# Autodesk Inventor assembly: 20mm Camera Rig Assmebly For Robot
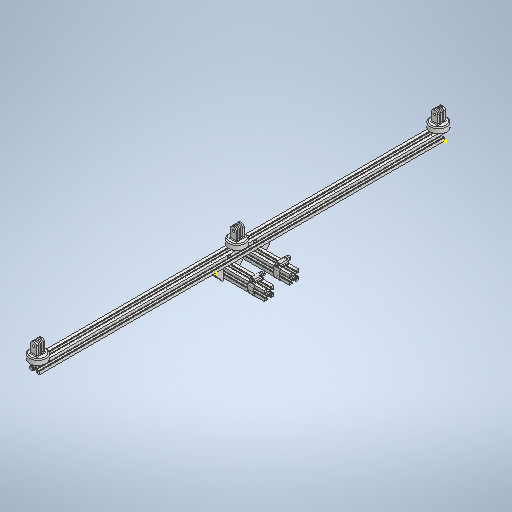
[picture p0: Inventor's stored thumbnail of the model, 512x512]
Saved by Autodesk Inventor 2025 (Build 290162010, 162A)
## iProperties
Created: 2024-07-24
Part Number: 20mm Camera Rig Assmebly For Robot
Document SubType Name: Assembly
Designer: Big Sean T
Author: Big Sean T
## Documents named in this file (9)
- D:\Underwater Camera RigScuba Resources\20mm Camera Rig Assmebly For Robot.iam
- D:\Underwater Camera RigScuba Resources\T slot beam 20mm.ipt
- D:\Underwater Camera RigScuba Resources\Go Pro Mount with threaded mount.ipt
- D:\Underwater Camera RigScuba Resources\M5 Model.ipt
- D:\Underwater Camera RigScuba Resources\90 Degree attachment T Slot.ipt
- D:\Underwater Camera RigScuba Resources\5mm Button Head Screw Botch.ipt
- D:\Underwater Camera RigScuba Resources\T slot beam 20mm Dist_40mm.ipt
- D:\Underwater Camera RigScuba Resources\25-40mm Worm Clamp Screw.ipt
- D:\Underwater Camera RigScuba Resources\25-40mm Worm Clamp.ipt
## Components (28 placed, 8 different names)
1. T slot beam 20mm:1 — Slider:1, Slider:2, Slider:3, Slider:8, Slider:43, Slider:44
2. Go Pro Mount with threaded mount:1 — Rotational:5
3. Go Pro Mount with threaded mount:2 — Rotational:3
4. Go Pro Mount with threaded mount:3 — Rotational:4
5. M5 Model:1 — Slider:1, Rotational:4
6. M5 Model:2 — Slider:3, Rotational:5
7. M5 Model:3 — Slider:2, Rotational:3
8. 90 Degree attachment T Slot:9 — Rigid:18, Rigid:19
9. 5mm Button Head Screw Botch:14 — Rigid:18, Slider:8, Slider:43
10. 5mm Button Head Screw Botch:15 — Rigid:19, Rigid:20
11. M5 Model:14
12. M5 Model:15 — Rigid:20, Slider:30
13. T slot beam 20mm Dist_40mm:1 — Slider:30, Planar:1
14. T slot beam 20mm Dist_40mm:3 — Slider:42, Slider:45, Planar:2
15. 90 Degree attachment T Slot:14
16. 5mm Button Head Screw Botch:24 — Slider:44
17. 5mm Button Head Screw Botch:25
18. M5 Model:24
19. M5 Model:25 — Slider:42
20. 90 Degree attachment T Slot:15
21. 5mm Button Head Screw Botch:26
22. 5mm Button Head Screw Botch:27
23. M5 Model:26
24. M5 Model:27 — Slider:45
25. 25-40mm Worm Clamp Screw:1 — Rigid:45
26. 25-40mm Worm Clamp:1 — Rigid:45, Planar:1
27. 25-40mm Worm Clamp Screw:3
28. 25-40mm Worm Clamp:3 — Planar:2
## Relationships (28: WeldJoint 14, TranslationJoint 9, RevoluteJoint 3, PlanarJoint 2)
- Slider:1 [TranslationJoint]: T slot beam 20mm:1 ↔ M5 Model:1
- Slider:2 [TranslationJoint]: T slot beam 20mm:1 ↔ M5 Model:3
- Slider:3 [TranslationJoint]: T slot beam 20mm:1 ↔ M5 Model:2
- Rotational:3 [RevoluteJoint]: Go Pro Mount with threaded mount:2 ↔ M5 Model:3
- Rotational:4 [RevoluteJoint]: Go Pro Mount with threaded mount:3 ↔ M5 Model:1
- Rotational:5 [RevoluteJoint]: Go Pro Mount with threaded mount:1 ↔ M5 Model:2
- Rigid:18 [WeldJoint]: 90 Degree attachment T Slot:9 ↔ 5mm Button Head Screw Botch:14
- Rigid:19 [WeldJoint]: 90 Degree attachment T Slot:9 ↔ 5mm Button Head Screw Botch:15
- [WeldJoint]: 5mm Button Head Screw Botch:14 ↔ M5 Model:14
- Rigid:20 [WeldJoint]: 5mm Button Head Screw Botch:15 ↔ M5 Model:15
- Slider:8 [TranslationJoint]: T slot beam 20mm:1 ↔ 5mm Button Head Screw Botch:14
- Slider:30 [TranslationJoint]: M5 Model:15 ↔ T slot beam 20mm Dist_40mm:1
- [WeldJoint]: 90 Degree attachment T Slot:14 ↔ 5mm Button Head Screw Botch:24
- [WeldJoint]: 90 Degree attachment T Slot:14 ↔ 5mm Button Head Screw Botch:25
- [WeldJoint]: 5mm Button Head Screw Botch:24 ↔ M5 Model:24
- [WeldJoint]: 5mm Button Head Screw Botch:25 ↔ M5 Model:25
- Slider:42 [TranslationJoint]: T slot beam 20mm Dist_40mm:3 ↔ M5 Model:25
- Slider:43 [TranslationJoint]: T slot beam 20mm:1 ↔ 5mm Button Head Screw Botch:14
- Slider:44 [TranslationJoint]: T slot beam 20mm:1 ↔ 5mm Button Head Screw Botch:24
- [WeldJoint]: 90 Degree attachment T Slot:15 ↔ 5mm Button Head Screw Botch:26
- [WeldJoint]: 90 Degree attachment T Slot:15 ↔ 5mm Button Head Screw Botch:27
- [WeldJoint]: 5mm Button Head Screw Botch:26 ↔ M5 Model:26
- [WeldJoint]: 5mm Button Head Screw Botch:27 ↔ M5 Model:27
- Slider:45 [TranslationJoint]: T slot beam 20mm Dist_40mm:3 ↔ M5 Model:27
- Rigid:45 [WeldJoint]: 25-40mm Worm Clamp Screw:1 ↔ 25-40mm Worm Clamp:1
- [WeldJoint]: 25-40mm Worm Clamp Screw:3 ↔ 25-40mm Worm Clamp:3
- Planar:1: T slot beam 20mm Dist_40mm:1 ↔ 25-40mm Worm Clamp:1
- Planar:2: T slot beam 20mm Dist_40mm:3 ↔ 25-40mm Worm Clamp:3
## Named parameters: d67_d46_d32 = 94.344904 deg, d68_d47_d33 = 0.23685 mm, d69_d48_d36 = 151.558906 deg, d70_d49_d37 = 21.01686 mm, d71_d50 = 0 mm, d72_d51 = 171.88213 deg, d73_d52 = -4.47026 mm, d185_d171_d67_d46_d32 = 94.344904 deg, d186_d172_d68_d47_d33 = 0.23685 mm, d187_d173_d69_d48_d36 = 151.558906 deg, d188_d174_d70_d49_d37 = 21.01686 mm, d189_d175_d71_d50 = 0 mm, d190_d176_d72_d51 = 171.88213 deg, d191_d177_d73_d52 = -4.47026 mm, d192_d178_d75 = 0 mm, d193_d179_d76 = 0 mm, d194_d180_d77 = 0 mm, d203_d185_d171_d67_d46_d32 = 94.344904 deg, d204_d186_d172_d68_d47_d33 = 0.23685 mm, d205_d187_d173_d69_d48_d36 = 151.558906 deg, d206_d188_d174_d70_d49_d37 = 21.01686 mm, d207_d189_d175_d71_d50 = 0 mm, d208_d190_d176_d72_d51 = 171.88213 deg, d209_d191_d177_d73_d52 = -4.47026 mm, d210_d192_d178_d75 = 0 mm, d211_d193_d179_d76 = 0 mm, d212_d194_d180_d77 = 0 mm, d216_d215 = 0 mm
